# Autodesk Inventor assembly: MARK3_Assembly
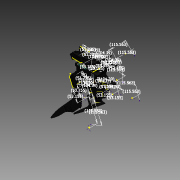
[picture p0: Inventor's stored thumbnail of the model, 180x180]
Saved by Autodesk Inventor 2014 SP2 (Build 180246200, 246)
## iProperties
Created: 2014-12-16
Part Number: MARK3_Assembly
Document SubType Name: Assembly
Designer: Sergei
Author: Sergei
## Documents named in this file (16)
- C:\Users\Sergei\Documents\Mini_Quad_Bot_Sergei_Dines\MARK 3\MARK3_Assembly.iam
- C:\Users\Sergei\Documents\raspberry-pi-model-b+\Imported Components\raspberrypi_b_+_(assembly)\raspberrypi_b_+_(assembly).iam
- C:\Users\Sergei\Documents\Mini_Quad_Bot_Sergei_Dines\MARK2\plate_mark2_sergeidines.ipt
- C:\Users\Sergei\Documents\Mini_Quad_Bot_Sergei_Dines\#4_0.25in_spacer.ipt
- C:\Users\Sergei\Documents\Mini_Quad_Bot_Sergei_Dines\MARK2\custom_spacer.ipt
- C:\Users\Sergei\Documents\Mini_Quad_Bot_Sergei_Dines\MARK2\plate_mark2_bracket_sergeidines.ipt
- C:\Users\Sergei\Documents\Mini_Quad_Bot_Sergei_Dines\MARK_1\small_L_micro_servo_bracket_sergei_dines.ipt
- C:\Users\Sergei\Documents\Mini_Quad_Bot_Sergei_Dines\MARK_1\#4_0.25In_Spacer_2.ipt
- C:\Users\Sergei\Documents\Mini_Quad_Bot_Sergei_Dines\MARK_1\micro_servo_bracket_sergei_dines.0015.ipt
- C:\Users\Sergei\Documents\Mini_Quad_Bot_Sergei_Dines\MARK_1\TOWERpro_MG90S_MicroServo-SD.ipt
- C:\Users\Sergei\Documents\Mini_Quad_Bot_Sergei_Dines\#4Bolt_0.5625in.ipt
- C:\Users\Sergei\Documents\Mini_Quad_Bot_Sergei_Dines\micro_servo_horn.ipt
- C:\Users\Sergei\Documents\Mini_Quad_Bot_Sergei_Dines\MARK 3\C_MARK3.ipt
- C:\Users\Sergei\Documents\Mini_Quad_Bot_Sergei_Dines\MARK 3\CLAW.ipt
- C:\Users\Sergei\Documents\Mini_Quad_Bot_Sergei_Dines\MARK 3\L_micro_sergei_dines.ipt
- C:\Users\Sergei\Documents\Mini_Quad_Bot_Sergei_Dines\MARK 3\multi_mark3_SergeiDines.ipt
## Components (67 placed, 15 different names)
1. raspberrypi_b_+_(assembly):1 [sub-assembly] — Mate:1, Mate:2, Mate:5, Mate:8, Mate:10, Mate:12, Mate:14, Mate:15, Mate:16, Mate:17, Mate:18, Mate:19, Mate:20, Mate:21
2. plate_mark2_sergeidines:1 — Mate:1, Mate:2, Mate:5, Mate:6, Mate:7, Mate:9, Mate:11, Mate:13
3. custom_spacer:2 — Mate:6, Mate:7
4. custom_spacer:3 — Mate:8, Mate:9
5. custom_spacer:4 — Mate:10, Mate:11
6. custom_spacer:5 — Mate:12, Mate:13
7. plate_mark2_bracket_sergeidines:1 — Mate:22, Mate:23, Mate:24, Mate:44, Mate:46, Mate:47, Mate:48, Mate:49, Mate:50, Mate:54, Mate:55, Mate:56, Mate:57, Mate:58, Mate:59, Mate:60, Mate:65, Mate:66, Mate:67, Mate:68, Mate:69, Mate:70, Mate:71, Mate:72
8. #4_0.25in_spacer:1 — Mate:17, Mate:20, Mate:22
9. #4_0.25in_spacer:2 — Mate:16, Mate:21
10. #4_0.25in_spacer:3 — Mate:14, Mate:18
11. #4_0.25in_spacer:4 — Mate:15, Mate:19, Mate:23, Mate:24
12. #4_0.25In_Spacer_2:2 — Mate:44, Mate:49, Mate:51, Mate:53
13. #4_0.25In_Spacer_2:3 — Mate:46, Mate:48, Mate:52
14. #4_0.25In_Spacer_2:4 — Mate:47, Mate:50
15. small_L_micro_servo_bracket_sergei_dines:9 — Mate:51, Mate:52, Mate:53, Mate:192, Mate:193, Mate:194
16. #4_0.25In_Spacer_2:5 — Mate:56, Mate:59, Mate:61, Mate:64
17. #4_0.25In_Spacer_2:6 — Mate:54, Mate:60, Mate:63
18. #4_0.25In_Spacer_2:7 — Mate:55
19. #4_0.25In_Spacer_2:8 — Mate:57, Mate:58, Mate:62
20. small_L_micro_servo_bracket_sergei_dines:10 — Mate:61, Mate:62, Mate:63, Mate:64, Mate:168, Mate:169, Mate:170
21. #4_0.25In_Spacer_2:9 — Mate:65, Mate:68, Mate:73
22. #4_0.25In_Spacer_2:10 — Mate:66, Mate:67, Mate:74, Mate:75
23. small_L_micro_servo_bracket_sergei_dines:11 — Mate:73, Mate:74, Mate:75, Mate:82, Mate:83, Mate:91
24. #4_0.25In_Spacer_2:11 — Mate:69, Mate:72, Mate:76
25. #4_0.25In_Spacer_2:12 — Mate:70, Mate:71, Mate:77, Mate:78
26. small_L_micro_servo_bracket_sergei_dines:12 — Mate:76, Mate:77, Mate:78, Mate:144, Mate:145, Mate:146
27. micro_servo_bracket_sergei_dines.0015:3 — Mate:82, Mate:83, Mate:91, Mate:92, Mate:93, Angle:1, Mate:94, Mate:95, Flush:1
28. TOWERpro_MG90S_MicroServo-SD:1 — Mate:92, Mate:93, Angle:1, Mate:96, Mate:97, Mate:98, Flush:1, Mate:231
29. #4Bolt_0.5625in:2 — Mate:94, Mate:95, Mate:96
30. TOWERpro_MG90S_MicroServo-SD:4 — Mate:117, Mate:118, Mate:119, Mate:238, Flush:6
31. micro_servo_horn:1 — Mate:97, Mate:98, Mate:232
32. micro_servo_bracket_sergei_dines.0015:8 — Mate:120, Mate:121, Mate:122, Mate:237, Mate:239, Mate:240, Mate:241
33. micro_servo_bracket_sergei_dines.0015:9 — Mate:117, Mate:118, Mate:119, Mate:233, Mate:234, Mate:235
34. TOWERpro_MG90S_MicroServo-SD:5 — Mate:120, Mate:121, Mate:122, Mate:236
35. micro_servo_bracket_sergei_dines.0015:10 — Mate:144, Mate:145, Mate:146, Mate:222, Mate:223, Mate:224, Angle:8
36. TOWERpro_MG90S_MicroServo-SD:6 — Mate:221, Mate:222
37. TOWERpro_MG90S_MicroServo-SD:7
38. small_L_micro_servo_bracket_sergei_dines:14 — Angle:7
39. micro_servo_horn:2
40. micro_servo_bracket_sergei_dines.0015:11 — Mate:229, Mate:230, Angle:9
41. micro_servo_bracket_sergei_dines.0015:12 — Mate:225, Mate:226, Mate:227, Angle:7
42. TOWERpro_MG90S_MicroServo-SD:8 — Mate:228
43. micro_servo_bracket_sergei_dines.0015:13 — Mate:168, Mate:169, Mate:170, Mate:214, Mate:215
44. TOWERpro_MG90S_MicroServo-SD:9 — Mate:213
45. TOWERpro_MG90S_MicroServo-SD:10
46. small_L_micro_servo_bracket_sergei_dines:15
47. micro_servo_horn:3
48. micro_servo_bracket_sergei_dines.0015:14 — Mate:220
49. micro_servo_bracket_sergei_dines.0015:15 — Mate:216, Mate:217, Mate:218
50. TOWERpro_MG90S_MicroServo-SD:11 — Mate:219
51. micro_servo_bracket_sergei_dines.0015:16 — Mate:192, Mate:193, Mate:194, Mate:196, Mate:197, Angle:5
52. TOWERpro_MG90S_MicroServo-SD:12 — Mate:195
53. TOWERpro_MG90S_MicroServo-SD:13 — Mate:203, Flush:5, Mate:207, Mate:208, Mate:209
54. micro_servo_horn:4
55. micro_servo_bracket_sergei_dines.0015:17 — Mate:202, Mate:210, Mate:211, Mate:212
56. TOWERpro_MG90S_MicroServo-SD:14 — Mate:201
57. C_MARK3:1 — Mate:195, Mate:196, Mate:197, Mate:204, Mate:205, Mate:206, Angle:5
58. CLAW:1 — Mate:201, Mate:202
59. L_micro_sergei_dines:2 — Mate:203, Flush:5, Mate:210, Mate:211, Mate:212, Angle:6
60. multi_mark3_SergeiDines:1 — Mate:204, Mate:205, Mate:206, Mate:207, Mate:208, Mate:209, Angle:6
61. C_MARK3:2 — Mate:213, Mate:214, Mate:215, Mate:216, Mate:217, Mate:218
62. CLAW:2 — Mate:219, Mate:220
63. C_MARK3:3 — Mate:221, Mate:223, Mate:224, Mate:225, Mate:226, Mate:227, Angle:8
64. CLAW:3 — Mate:228, Mate:229, Mate:230, Angle:9
65. C_MARK3:4 — Mate:231, Mate:232, Mate:233, Mate:234, Mate:235
66. CLAW:4 — Mate:236, Mate:237
67. L_micro_sergei_dines:3 — Mate:238, Flush:6, Mate:239, Mate:240, Mate:241
## Relationships (177: Mate 162, Angle 9, Flush 6)
- Mate:1: raspberrypi_b_+_(assembly):1 ↔ plate_mark2_sergeidines:1
- Mate:2: raspberrypi_b_+_(assembly):1 ↔ plate_mark2_sergeidines:1
- Mate:5: raspberrypi_b_+_(assembly):1 ↔ plate_mark2_sergeidines:1
- Mate:6: plate_mark2_sergeidines:1 ↔ custom_spacer:2
- Mate:7: plate_mark2_sergeidines:1 ↔ custom_spacer:2
- Mate:8: raspberrypi_b_+_(assembly):1 ↔ custom_spacer:3
- Mate:9: plate_mark2_sergeidines:1 ↔ custom_spacer:3
- Mate:10: raspberrypi_b_+_(assembly):1 ↔ custom_spacer:4
- Mate:11: plate_mark2_sergeidines:1 ↔ custom_spacer:4
- Mate:12: raspberrypi_b_+_(assembly):1 ↔ custom_spacer:5
- Mate:13: plate_mark2_sergeidines:1 ↔ custom_spacer:5
- Mate:14: raspberrypi_b_+_(assembly):1 ↔ #4_0.25in_spacer:3
- Mate:15: raspberrypi_b_+_(assembly):1 ↔ #4_0.25in_spacer:4
- Mate:16: raspberrypi_b_+_(assembly):1 ↔ #4_0.25in_spacer:2
- Mate:17: raspberrypi_b_+_(assembly):1 ↔ #4_0.25in_spacer:1
- Mate:18: raspberrypi_b_+_(assembly):1 ↔ #4_0.25in_spacer:3
- Mate:19: raspberrypi_b_+_(assembly):1 ↔ #4_0.25in_spacer:4
- Mate:20: raspberrypi_b_+_(assembly):1 ↔ #4_0.25in_spacer:1
- Mate:21: raspberrypi_b_+_(assembly):1 ↔ #4_0.25in_spacer:2
- Mate:22: plate_mark2_bracket_sergeidines:1 ↔ #4_0.25in_spacer:1
- Mate:23: plate_mark2_bracket_sergeidines:1 ↔ #4_0.25in_spacer:4
- Mate:24: plate_mark2_bracket_sergeidines:1 ↔ #4_0.25in_spacer:4
- Mate:44: plate_mark2_bracket_sergeidines:1 ↔ #4_0.25In_Spacer_2:2
- Mate:46: plate_mark2_bracket_sergeidines:1 ↔ #4_0.25In_Spacer_2:3
- Mate:47: plate_mark2_bracket_sergeidines:1 ↔ #4_0.25In_Spacer_2:4
- Mate:48: plate_mark2_bracket_sergeidines:1 ↔ #4_0.25In_Spacer_2:3
- Mate:49: plate_mark2_bracket_sergeidines:1 ↔ #4_0.25In_Spacer_2:2
- Mate:50: plate_mark2_bracket_sergeidines:1 ↔ #4_0.25In_Spacer_2:4
- Mate:51: #4_0.25In_Spacer_2:2 ↔ small_L_micro_servo_bracket_sergei_dines:9
- Mate:52: #4_0.25In_Spacer_2:3 ↔ small_L_micro_servo_bracket_sergei_dines:9
- Mate:53: #4_0.25In_Spacer_2:2 ↔ small_L_micro_servo_bracket_sergei_dines:9
- Mate:54: plate_mark2_bracket_sergeidines:1 ↔ #4_0.25In_Spacer_2:6
- Mate:55: plate_mark2_bracket_sergeidines:1 ↔ #4_0.25In_Spacer_2:7
- Mate:56: plate_mark2_bracket_sergeidines:1 ↔ #4_0.25In_Spacer_2:5
- Mate:57: plate_mark2_bracket_sergeidines:1 ↔ #4_0.25In_Spacer_2:8
- Mate:58: plate_mark2_bracket_sergeidines:1 ↔ #4_0.25In_Spacer_2:8
- Mate:59: plate_mark2_bracket_sergeidines:1 ↔ #4_0.25In_Spacer_2:5
- Mate:60: plate_mark2_bracket_sergeidines:1 ↔ #4_0.25In_Spacer_2:6
- Mate:61: #4_0.25In_Spacer_2:5 ↔ small_L_micro_servo_bracket_sergei_dines:10
- Mate:62: #4_0.25In_Spacer_2:8 ↔ small_L_micro_servo_bracket_sergei_dines:10
- Mate:63: #4_0.25In_Spacer_2:6 ↔ small_L_micro_servo_bracket_sergei_dines:10
- Mate:64: #4_0.25In_Spacer_2:5 ↔ small_L_micro_servo_bracket_sergei_dines:10
- Mate:65: plate_mark2_bracket_sergeidines:1 ↔ #4_0.25In_Spacer_2:9
- Mate:66: plate_mark2_bracket_sergeidines:1 ↔ #4_0.25In_Spacer_2:10
- Mate:67: plate_mark2_bracket_sergeidines:1 ↔ #4_0.25In_Spacer_2:10
- Mate:68: plate_mark2_bracket_sergeidines:1 ↔ #4_0.25In_Spacer_2:9
- Mate:69: plate_mark2_bracket_sergeidines:1 ↔ #4_0.25In_Spacer_2:11
- Mate:70: plate_mark2_bracket_sergeidines:1 ↔ #4_0.25In_Spacer_2:12
- Mate:71: plate_mark2_bracket_sergeidines:1 ↔ #4_0.25In_Spacer_2:12
- Mate:72: plate_mark2_bracket_sergeidines:1 ↔ #4_0.25In_Spacer_2:11
- Mate:73: #4_0.25In_Spacer_2:9 ↔ small_L_micro_servo_bracket_sergei_dines:11
- Mate:74: #4_0.25In_Spacer_2:10 ↔ small_L_micro_servo_bracket_sergei_dines:11
- Mate:75: #4_0.25In_Spacer_2:10 ↔ small_L_micro_servo_bracket_sergei_dines:11
- Mate:76: #4_0.25In_Spacer_2:11 ↔ small_L_micro_servo_bracket_sergei_dines:12
- Mate:77: #4_0.25In_Spacer_2:12 ↔ small_L_micro_servo_bracket_sergei_dines:12
- Mate:78: #4_0.25In_Spacer_2:12 ↔ small_L_micro_servo_bracket_sergei_dines:12
- Mate:82: small_L_micro_servo_bracket_sergei_dines:11 ↔ micro_servo_bracket_sergei_dines.0015:3
- Mate:83: small_L_micro_servo_bracket_sergei_dines:11 ↔ micro_servo_bracket_sergei_dines.0015:3
- Mate:91: small_L_micro_servo_bracket_sergei_dines:11 ↔ micro_servo_bracket_sergei_dines.0015:3
- Mate:92: micro_servo_bracket_sergei_dines.0015:3 ↔ TOWERpro_MG90S_MicroServo-SD:1
- Mate:93: micro_servo_bracket_sergei_dines.0015:3 ↔ TOWERpro_MG90S_MicroServo-SD:1
- Angle:1 (0 deg): micro_servo_bracket_sergei_dines.0015:3 ↔ TOWERpro_MG90S_MicroServo-SD:1
- Mate:94: micro_servo_bracket_sergei_dines.0015:3 ↔ #4Bolt_0.5625in:2
- Mate:95: micro_servo_bracket_sergei_dines.0015:3 ↔ #4Bolt_0.5625in:2
- Mate:96: TOWERpro_MG90S_MicroServo-SD:1 ↔ #4Bolt_0.5625in:2
- Mate:97: TOWERpro_MG90S_MicroServo-SD:1 ↔ micro_servo_horn:1
- Mate:98: TOWERpro_MG90S_MicroServo-SD:1 ↔ micro_servo_horn:1
- Flush:1: micro_servo_bracket_sergei_dines.0015:3 ↔ TOWERpro_MG90S_MicroServo-SD:1
- Mate:117: TOWERpro_MG90S_MicroServo-SD:4 ↔ micro_servo_bracket_sergei_dines.0015:9
- Mate:118: TOWERpro_MG90S_MicroServo-SD:4 ↔ micro_servo_bracket_sergei_dines.0015:9
- Mate:119: TOWERpro_MG90S_MicroServo-SD:4 ↔ micro_servo_bracket_sergei_dines.0015:9
- Mate:120: micro_servo_bracket_sergei_dines.0015:8 ↔ TOWERpro_MG90S_MicroServo-SD:5
- Mate:121: micro_servo_bracket_sergei_dines.0015:8 ↔ TOWERpro_MG90S_MicroServo-SD:5
- Mate:122: micro_servo_bracket_sergei_dines.0015:8 ↔ TOWERpro_MG90S_MicroServo-SD:5
- [Mate]: micro_servo_bracket_sergei_dines.0015:10 ↔ TOWERpro_MG90S_MicroServo-SD:6
- [Mate]: micro_servo_bracket_sergei_dines.0015:10 ↔ TOWERpro_MG90S_MicroServo-SD:6
- [Angle] (0 deg): micro_servo_bracket_sergei_dines.0015:10 ↔ TOWERpro_MG90S_MicroServo-SD:6
- [Mate]: TOWERpro_MG90S_MicroServo-SD:6 ↔ micro_servo_horn:2
- [Mate]: TOWERpro_MG90S_MicroServo-SD:6 ↔ micro_servo_horn:2
- [Flush]: micro_servo_bracket_sergei_dines.0015:10 ↔ TOWERpro_MG90S_MicroServo-SD:6
- [Mate]: TOWERpro_MG90S_MicroServo-SD:7 ↔ small_L_micro_servo_bracket_sergei_dines:14
- [Mate]: TOWERpro_MG90S_MicroServo-SD:7 ↔ small_L_micro_servo_bracket_sergei_dines:14
- [Mate]: small_L_micro_servo_bracket_sergei_dines:14 ↔ micro_servo_bracket_sergei_dines.0015:11
- [Mate]: small_L_micro_servo_bracket_sergei_dines:14 ↔ micro_servo_bracket_sergei_dines.0015:11
- [Mate]: small_L_micro_servo_bracket_sergei_dines:14 ↔ micro_servo_bracket_sergei_dines.0015:11
- [Mate]: TOWERpro_MG90S_MicroServo-SD:7 ↔ micro_servo_bracket_sergei_dines.0015:12
- [Mate]: TOWERpro_MG90S_MicroServo-SD:7 ↔ micro_servo_bracket_sergei_dines.0015:12
- [Mate]: TOWERpro_MG90S_MicroServo-SD:7 ↔ micro_servo_bracket_sergei_dines.0015:12
- [Mate]: micro_servo_bracket_sergei_dines.0015:11 ↔ TOWERpro_MG90S_MicroServo-SD:8
- [Mate]: micro_servo_bracket_sergei_dines.0015:11 ↔ TOWERpro_MG90S_MicroServo-SD:8
- [Mate]: micro_servo_bracket_sergei_dines.0015:11 ↔ TOWERpro_MG90S_MicroServo-SD:8
- Mate:144: small_L_micro_servo_bracket_sergei_dines:12 ↔ micro_servo_bracket_sergei_dines.0015:10
- Mate:145: small_L_micro_servo_bracket_sergei_dines:12 ↔ micro_servo_bracket_sergei_dines.0015:10
- Mate:146: small_L_micro_servo_bracket_sergei_dines:12 ↔ micro_servo_bracket_sergei_dines.0015:10
- [Mate]: micro_servo_bracket_sergei_dines.0015:13 ↔ TOWERpro_MG90S_MicroServo-SD:9
- [Mate]: micro_servo_bracket_sergei_dines.0015:13 ↔ TOWERpro_MG90S_MicroServo-SD:9
- [Angle] (0 deg): micro_servo_bracket_sergei_dines.0015:13 ↔ TOWERpro_MG90S_MicroServo-SD:9
- [Mate]: TOWERpro_MG90S_MicroServo-SD:9 ↔ micro_servo_horn:3
- [Mate]: TOWERpro_MG90S_MicroServo-SD:9 ↔ micro_servo_horn:3
- [Flush]: micro_servo_bracket_sergei_dines.0015:13 ↔ TOWERpro_MG90S_MicroServo-SD:9
- [Mate]: TOWERpro_MG90S_MicroServo-SD:10 ↔ small_L_micro_servo_bracket_sergei_dines:15
- [Mate]: TOWERpro_MG90S_MicroServo-SD:10 ↔ small_L_micro_servo_bracket_sergei_dines:15
- [Mate]: small_L_micro_servo_bracket_sergei_dines:15 ↔ micro_servo_bracket_sergei_dines.0015:14
- [Mate]: small_L_micro_servo_bracket_sergei_dines:15 ↔ micro_servo_bracket_sergei_dines.0015:14
- [Mate]: small_L_micro_servo_bracket_sergei_dines:15 ↔ micro_servo_bracket_sergei_dines.0015:14
- [Mate]: TOWERpro_MG90S_MicroServo-SD:10 ↔ micro_servo_bracket_sergei_dines.0015:15
- [Mate]: TOWERpro_MG90S_MicroServo-SD:10 ↔ micro_servo_bracket_sergei_dines.0015:15
- [Mate]: TOWERpro_MG90S_MicroServo-SD:10 ↔ micro_servo_bracket_sergei_dines.0015:15
- [Mate]: micro_servo_bracket_sergei_dines.0015:14 ↔ TOWERpro_MG90S_MicroServo-SD:11
- [Mate]: micro_servo_bracket_sergei_dines.0015:14 ↔ TOWERpro_MG90S_MicroServo-SD:11
- [Mate]: micro_servo_bracket_sergei_dines.0015:14 ↔ TOWERpro_MG90S_MicroServo-SD:11
- Mate:168: small_L_micro_servo_bracket_sergei_dines:10 ↔ micro_servo_bracket_sergei_dines.0015:13
- Mate:169: small_L_micro_servo_bracket_sergei_dines:10 ↔ micro_servo_bracket_sergei_dines.0015:13
- Mate:170: small_L_micro_servo_bracket_sergei_dines:10 ↔ micro_servo_bracket_sergei_dines.0015:13
- [Mate]: micro_servo_bracket_sergei_dines.0015:16 ↔ TOWERpro_MG90S_MicroServo-SD:12
- [Mate]: micro_servo_bracket_sergei_dines.0015:16 ↔ TOWERpro_MG90S_MicroServo-SD:12
- [Angle] (0 deg): micro_servo_bracket_sergei_dines.0015:16 ↔ TOWERpro_MG90S_MicroServo-SD:12
- [Mate]: TOWERpro_MG90S_MicroServo-SD:12 ↔ micro_servo_horn:4
- [Mate]: TOWERpro_MG90S_MicroServo-SD:12 ↔ micro_servo_horn:4
- [Flush]: micro_servo_bracket_sergei_dines.0015:16 ↔ TOWERpro_MG90S_MicroServo-SD:12
- [Mate]: micro_servo_bracket_sergei_dines.0015:17 ↔ TOWERpro_MG90S_MicroServo-SD:14
- [Mate]: micro_servo_bracket_sergei_dines.0015:17 ↔ TOWERpro_MG90S_MicroServo-SD:14
- [Mate]: micro_servo_bracket_sergei_dines.0015:17 ↔ TOWERpro_MG90S_MicroServo-SD:14
- Mate:192: small_L_micro_servo_bracket_sergei_dines:9 ↔ micro_servo_bracket_sergei_dines.0015:16
- Mate:193: small_L_micro_servo_bracket_sergei_dines:9 ↔ micro_servo_bracket_sergei_dines.0015:16
- Mate:194: small_L_micro_servo_bracket_sergei_dines:9 ↔ micro_servo_bracket_sergei_dines.0015:16
- Mate:195: TOWERpro_MG90S_MicroServo-SD:12 ↔ C_MARK3:1
- Mate:196: micro_servo_bracket_sergei_dines.0015:16 ↔ C_MARK3:1
- Mate:197: micro_servo_bracket_sergei_dines.0015:16 ↔ C_MARK3:1
- Mate:201: TOWERpro_MG90S_MicroServo-SD:14 ↔ CLAW:1
- Mate:202: micro_servo_bracket_sergei_dines.0015:17 ↔ CLAW:1
- Mate:203: TOWERpro_MG90S_MicroServo-SD:13 ↔ L_micro_sergei_dines:2
- Flush:5: TOWERpro_MG90S_MicroServo-SD:13 ↔ L_micro_sergei_dines:2
- Mate:204: C_MARK3:1 ↔ multi_mark3_SergeiDines:1
- Mate:205: C_MARK3:1 ↔ multi_mark3_SergeiDines:1
- Mate:206: C_MARK3:1 ↔ multi_mark3_SergeiDines:1
- Mate:207: TOWERpro_MG90S_MicroServo-SD:13 ↔ multi_mark3_SergeiDines:1
- Mate:208: TOWERpro_MG90S_MicroServo-SD:13 ↔ multi_mark3_SergeiDines:1
- Mate:209: TOWERpro_MG90S_MicroServo-SD:13 ↔ multi_mark3_SergeiDines:1
- Angle:5 (438 deg): micro_servo_bracket_sergei_dines.0015:16 ↔ C_MARK3:1
- Mate:210: micro_servo_bracket_sergei_dines.0015:17 ↔ L_micro_sergei_dines:2
- Mate:211: micro_servo_bracket_sergei_dines.0015:17 ↔ L_micro_sergei_dines:2
- Mate:212: micro_servo_bracket_sergei_dines.0015:17 ↔ L_micro_sergei_dines:2
- Angle:6 (120 deg): L_micro_sergei_dines:2 ↔ multi_mark3_SergeiDines:1
- Mate:213: TOWERpro_MG90S_MicroServo-SD:9 ↔ C_MARK3:2
- Mate:214: micro_servo_bracket_sergei_dines.0015:13 ↔ C_MARK3:2
- Mate:215: micro_servo_bracket_sergei_dines.0015:13 ↔ C_MARK3:2
- Mate:216: micro_servo_bracket_sergei_dines.0015:15 ↔ C_MARK3:2
- Mate:217: micro_servo_bracket_sergei_dines.0015:15 ↔ C_MARK3:2
- Mate:218: micro_servo_bracket_sergei_dines.0015:15 ↔ C_MARK3:2
- Mate:219: TOWERpro_MG90S_MicroServo-SD:11 ↔ CLAW:2
- Mate:220: micro_servo_bracket_sergei_dines.0015:14 ↔ CLAW:2
- Mate:221: TOWERpro_MG90S_MicroServo-SD:6 ↔ C_MARK3:3
- Mate:222: micro_servo_bracket_sergei_dines.0015:10 ↔ TOWERpro_MG90S_MicroServo-SD:6
- Mate:223: micro_servo_bracket_sergei_dines.0015:10 ↔ C_MARK3:3
- Mate:224: micro_servo_bracket_sergei_dines.0015:10 ↔ C_MARK3:3
- Mate:225: micro_servo_bracket_sergei_dines.0015:12 ↔ C_MARK3:3
- Mate:226: micro_servo_bracket_sergei_dines.0015:12 ↔ C_MARK3:3
- Mate:227: micro_servo_bracket_sergei_dines.0015:12 ↔ C_MARK3:3
- Mate:228: TOWERpro_MG90S_MicroServo-SD:8 ↔ CLAW:3
- Mate:229: micro_servo_bracket_sergei_dines.0015:11 ↔ CLAW:3
- Mate:230: micro_servo_bracket_sergei_dines.0015:11 ↔ CLAW:3
- Mate:231: TOWERpro_MG90S_MicroServo-SD:1 ↔ C_MARK3:4
- Mate:232: micro_servo_horn:1 ↔ C_MARK3:4
- Mate:233: micro_servo_bracket_sergei_dines.0015:9 ↔ C_MARK3:4
- Mate:234: micro_servo_bracket_sergei_dines.0015:9 ↔ C_MARK3:4
- Mate:235: micro_servo_bracket_sergei_dines.0015:9 ↔ C_MARK3:4
- Mate:236: TOWERpro_MG90S_MicroServo-SD:5 ↔ CLAW:4
- Mate:237: micro_servo_bracket_sergei_dines.0015:8 ↔ CLAW:4
- Mate:238: TOWERpro_MG90S_MicroServo-SD:4 ↔ L_micro_sergei_dines:3
- Flush:6: TOWERpro_MG90S_MicroServo-SD:4 ↔ L_micro_sergei_dines:3
- Mate:239: micro_servo_bracket_sergei_dines.0015:8 ↔ L_micro_sergei_dines:3
- Mate:240: micro_servo_bracket_sergei_dines.0015:8 ↔ L_micro_sergei_dines:3
- Mate:241: micro_servo_bracket_sergei_dines.0015:8 ↔ L_micro_sergei_dines:3
- Angle:7 (180 deg): small_L_micro_servo_bracket_sergei_dines:14 ↔ micro_servo_bracket_sergei_dines.0015:12
- Angle:8 (59 deg): micro_servo_bracket_sergei_dines.0015:10 ↔ C_MARK3:3
- Angle:9 (0 deg): micro_servo_bracket_sergei_dines.0015:11 ↔ CLAW:3
## Named parameters: d157_d146 = 0 mm, d158_d147 = 0 mm, d162_d151 = 0 mm, d163_d152 = 0 mm, d164_d153 = 0 mm, d165_d154 = 0 mm, d166_d155 = 0 mm, d167_d156 = 0 mm, d168_d121 = 0 mm, d169_d122 = 0 mm, d170_d123 = 0 mm, d174_d143 = 0 mm, d175_d144 = 0 mm, d176_d145 = 0 mm, d177_d113 = 0 mm, d178_d114 = 0 mm, d179_d115 = 0 deg, d183_d157_d146 = 0 mm, d184_d158_d147 = 0 mm, d188_d162_d151 = 0 mm, d189_d163_d152 = 0 mm, d190_d164_d153 = 0 mm, d191_d165_d154 = 0 mm, d192_d166_d155 = 0 mm, d193_d167_d156 = 0 mm, d194_d168_d121 = 0 mm, d195_d169_d122 = 0 mm, d196_d170_d123 = 0 mm, d200_d174_d143 = 0 mm, d201_d175_d144 = 0 mm, d202_d176_d145 = 0 mm, d203_d177_d113 = 0 mm, d204_d178_d114 = 0 mm, d205_d179_d115 = 0 deg, d217_d154 = 0 mm, d218_d155 = 0 mm, d219_d156 = 0 mm, d220_d121 = 0 mm, d221_d122 = 0 mm, d222_d123 = 0 mm, d229_d113 = 0 mm, d230_d114 = 0 mm, d231_d115 = 0 deg
